# Autodesk Inventor assembly: master_assembly_1
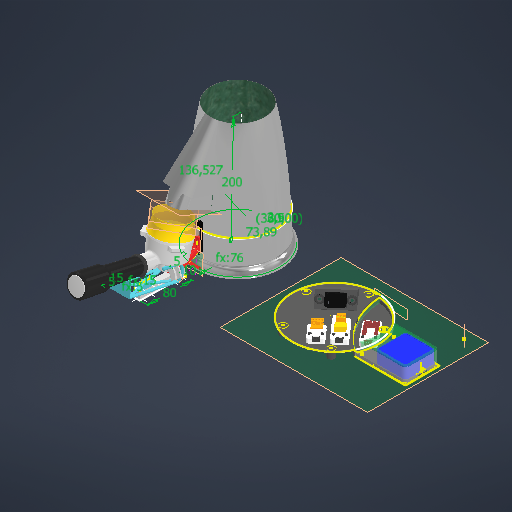
[picture p0: Inventor's stored thumbnail of the model, 512x512]
Saved by Autodesk Inventor 2026 (Build 300175000, 175)
## iProperties
Created: 2025-05-05
Part Number: master_assembly_1
Document SubType Name: Assembly
Designer: Paul Juschitz
Author: Paul Juschitz
## Documents named in this file (15)
- C:\Users\Paul Juschitz\Documents\private\m2m_GBW_mod\CAD\master\master_assembly.iam
- C:\Users\Paul Juschitz\Documents\private\m2m_GBW_mod\CAD\master\m2m_shell.ipt
- C:\Users\Paul Juschitz\Documents\private\m2m_GBW_mod\CAD\master\m2m_bottom.ipt
- C:\Users\Paul Juschitz\Documents\private\m2m_GBW_mod\CAD\master\load_cell.ipt
- C:\Users\Paul Juschitz\Documents\private\m2m_GBW_mod\CAD\master\BES870XL Portafilter\BES870XL Portafilter_assembled.iam
- C:\Users\Paul Juschitz\Documents\private\m2m_GBW_mod\CAD\master\mock_dosing_funnel.ipt
- C:\Users\Paul Juschitz\Documents\private\m2m_GBW_mod\CAD\master\load_cell_holder.ipt
- C:\Users\Paul Juschitz\Documents\private\m2m_GBW_mod\CAD\master\core_dummy.ipt
- C:\Users\Paul Juschitz\Documents\private\m2m_GBW_mod\CAD\master\my_portafilter_holder.ipt
- C:\Users\Paul Juschitz\Documents\private\m2m_GBW_mod\CAD\master\bottom_replacement_housing_bottom.ipt
- C:\Users\Paul Juschitz\Documents\private\m2m_GBW_mod\CAD\master\bottom_replacement_housing_top.ipt
- C:\Users\Paul Juschitz\Documents\private\m2m_GBW_mod\CAD\master\Mini_3A_Relay_Unit.iam
- C:\Users\Paul Juschitz\Documents\private\m2m_GBW_mod\CAD\master\Mini_Weight_Unit_HX711.iam
- C:\Users\Paul Juschitz\Documents\private\m2m_GBW_mod\CAD\master\PaHub_I2C_UNIT.iam
- C:\Users\Paul Juschitz\Documents\private\m2m_GBW_mod\CAD\master\my_C14.ipt
## Components (14 placed, 14 different names)
1. m2m_shell:1 — Mate:1, Mate:2, Mate:3, Mate:7, Tangent:3
2. m2m_bottom:1 — Mate:2, Mate:3, Flush:6
3. load_cell:1 — Mate:18, Cylindrical:9, Cylindrical:10, Mate:33
4. BES870XL Portafilter_assembled:1 [sub-assembly] — Mate:4, Tangent:4, Tangent:5, Mate:34, Cylindrical:11, Tangent:6
5. mock_dosing_funnel:1 — Cylindrical:11, Tangent:6
6. load_cell_holder:1 — Mate:7, Tangent:3, Mate:18, Cylindrical:9
7. core_dummy:1 — Mate:21, Mate:22
8. my_portafilter_holder:1 — Cylindrical:10, Mate:33, Tangent:4, Tangent:5, Mate:34
9. bottom_replacement_housing_bottom:1 — Mate:21, Mate:22, Mate:23, Mate:24, Mate:26, Cylindrical:1, Cylindrical:2, Mate:29, Mate:30, Cylindrical:3, Cylindrical:4, Mate:31, Mate:32, Cylindrical:5, Cylindrical:6, Cylindrical:7, Cylindrical:8
10. bottom_replacement_housing_top:1 — Mate:23, Mate:24
11. Mini_3A_Relay_Unit:1 [sub-assembly] — Mate:26, Mate:32, Cylindrical:6, Cylindrical:7
12. Mini_Weight_Unit_HX711:1 [sub-assembly] — Mate:31, Cylindrical:5, Cylindrical:8
13. PaHub_I2C_UNIT:1 [sub-assembly] — Mate:30, Cylindrical:3, Cylindrical:4
14. my_C14:1 — Cylindrical:1, Cylindrical:2, Mate:29
## Relationships (33: Mate 17, CylindricalJoint 11, Tangent 4, Flush 1)
- Mate:1: m2m_shell:1
- Mate:2: m2m_shell:1 ↔ m2m_bottom:1
- Mate:3: m2m_shell:1 ↔ m2m_bottom:1
- Mate:4: BES870XL Portafilter_assembled:1
- Mate:7: m2m_shell:1 ↔ load_cell_holder:1
- Tangent:3: m2m_shell:1 ↔ load_cell_holder:1
- Mate:18: load_cell:1 ↔ load_cell_holder:1
- Flush:6: m2m_bottom:1
- Mate:21: core_dummy:1 ↔ bottom_replacement_housing_bottom:1
- Mate:22: core_dummy:1 ↔ bottom_replacement_housing_bottom:1
- Mate:23: bottom_replacement_housing_bottom:1 ↔ bottom_replacement_housing_top:1
- Mate:24: bottom_replacement_housing_bottom:1 ↔ bottom_replacement_housing_top:1
- Mate:26: bottom_replacement_housing_bottom:1 ↔ Mini_3A_Relay_Unit:1
- Cylindrical:1: bottom_replacement_housing_bottom:1 ↔ my_C14:1
- Cylindrical:2: bottom_replacement_housing_bottom:1 ↔ my_C14:1
- Mate:29: bottom_replacement_housing_bottom:1 ↔ my_C14:1
- Mate:30: bottom_replacement_housing_bottom:1 ↔ PaHub_I2C_UNIT:1
- Cylindrical:3: bottom_replacement_housing_bottom:1 ↔ PaHub_I2C_UNIT:1
- Cylindrical:4: bottom_replacement_housing_bottom:1 ↔ PaHub_I2C_UNIT:1
- Mate:31: bottom_replacement_housing_bottom:1 ↔ Mini_Weight_Unit_HX711:1
- Mate:32: bottom_replacement_housing_bottom:1 ↔ Mini_3A_Relay_Unit:1
- Cylindrical:5: bottom_replacement_housing_bottom:1 ↔ Mini_Weight_Unit_HX711:1
- Cylindrical:6: bottom_replacement_housing_bottom:1 ↔ Mini_3A_Relay_Unit:1
- Cylindrical:7: bottom_replacement_housing_bottom:1 ↔ Mini_3A_Relay_Unit:1
- Cylindrical:8: bottom_replacement_housing_bottom:1 ↔ Mini_Weight_Unit_HX711:1
- Cylindrical:9: load_cell:1 ↔ load_cell_holder:1
- Cylindrical:10: load_cell:1 ↔ my_portafilter_holder:1
- Mate:33: load_cell:1 ↔ my_portafilter_holder:1
- Tangent:4: BES870XL Portafilter_assembled:1 ↔ my_portafilter_holder:1
- Tangent:5: BES870XL Portafilter_assembled:1 ↔ my_portafilter_holder:1
- Mate:34: BES870XL Portafilter_assembled:1 ↔ my_portafilter_holder:1
- Cylindrical:11: BES870XL Portafilter_assembled:1 ↔ mock_dosing_funnel:1
- Tangent:6: BES870XL Portafilter_assembled:1 ↔ mock_dosing_funnel:1
## Named parameters: m2m_bottom_radius_lower = 76 mm, m2m_bottom_radius_upper = 68 mm, m2m_top_radius = 48 mm, m2m_shell_thickness = 0.5 mm, m2m_shell_height = 220 mm, m2m_shell_base_height = 16 mm, m2m_shell_bottom_screwhole_inset = -2 mm, m2m_shell_bottom_screwhole_ID = 2.5 mm, m2m_shell_bottom_screwhole_OD = 3.9 mm, m2m_spout_height_inner = 93 mm, m2m_spout_height_outer = 121 mm, m2m_spout_angle = 27.5 deg, m2m_opening_bracket_outer_width = 20 mm, m2m_center_radius = 136.52735 mm, m2m_fork_bracket_outer_thickness = 3.8 mm, m2m_fork_bracket_inner_thickness = 0 mm, m2m_fork_bracket_height_bottom = 20.6 mm, m2m_fork_bracket_height = 50.4 mm, m2m_shell_spout_diameter = 30.6 mm
